# Autodesk Inventor assembly: Slead_Assemblie
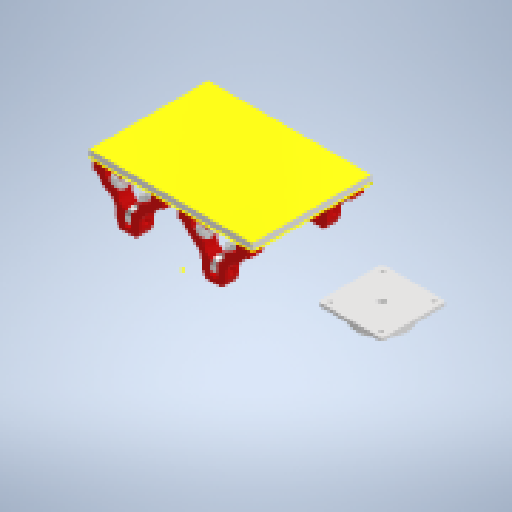
[picture p0: Inventor's stored thumbnail of the model, 512x512]
Saved by Autodesk Inventor 2024 (Build 280153000, 153)
## iProperties
Created: 2023-11-24
Part Number: Slead_Assemblie
Document SubType Name: Assembly
Designer: danie
Author: danie
## Documents named in this file (6)
- C:\GitHubDesktop\3d-model\basis_roboter\low_rider_v2\custom_files\Slead_Assemblie.iam
- C:\GitHubDesktop\3d-model\basis_roboter\low_rider_v2\custom_files\LR2_Assemblie.iam
- C:\GitHubDesktop\3d-model\basis_roboter\low_rider_v2\custom_files\Sleed_Plate.ipt
- C:\GitHubDesktop\3d-model\basis_roboter\Saugknopf.ipt
- C:\Users\danie\OneDrive\Documents\Inventor\Content Center Files\R2024\en-US\ISO 4017(1)\ISO 4017 - M5 x 20 - ISO.ipt
- C:\Users\danie\OneDrive\Documents\Inventor\Content Center Files\R2024\en-US\ISO 4035(2)\ISO 4035 - M5 - ISO.ipt
## Components (8 placed, 5 different names)
1. LR2_Assemblie:1 [sub-assembly] — Flush:1, Rigid:2
2. LR2_Assemblie:2 [sub-assembly] — Flush:3, Rigid:3
3. LR2_Assemblie:3 [sub-assembly] — Flush:2, Rigid:4
4. LR2_Assemblie:4 [sub-assembly] — Flush:4, Rigid:1
5. Sleed_Plate:1 — Flush:5, Rigid:1, Rigid:2, Rigid:3, Rigid:4, Rotational:1, Mate:4
6. Saugknopf:1 — Rotational:1, Mate:1, Mate:2, Mate:3
7. ISO 4017 M5 x 20:1 — Mate:1, Mate:2
8. ISO 4035 M5:1 — Mate:3, Mate:4
## Relationships (14: Flush 5, WeldJoint 4, Mate 4, RevoluteJoint 1)
- Flush:1: LR2_Assemblie:1
- Flush:2: LR2_Assemblie:3
- Flush:3: LR2_Assemblie:2
- Flush:4: LR2_Assemblie:4
- Flush:5: Sleed_Plate:1
- Rigid:1 [WeldJoint]: LR2_Assemblie:4 ↔ Sleed_Plate:1
- Rigid:2 [WeldJoint]: LR2_Assemblie:1 ↔ Sleed_Plate:1
- Rigid:3 [WeldJoint]: LR2_Assemblie:2 ↔ Sleed_Plate:1
- Rigid:4 [WeldJoint]: LR2_Assemblie:3 ↔ Sleed_Plate:1
- Rotational:1 [RevoluteJoint]: Sleed_Plate:1 ↔ Saugknopf:1
- Mate:1: Saugknopf:1 ↔ ISO 4017 M5 x 20:1
- Mate:2: Saugknopf:1 ↔ ISO 4017 M5 x 20:1
- Mate:3: Saugknopf:1 ↔ ISO 4035 M5:1
- Mate:4: Sleed_Plate:1 ↔ ISO 4035 M5:1
